# Autodesk Inventor assembly: motor_assembly
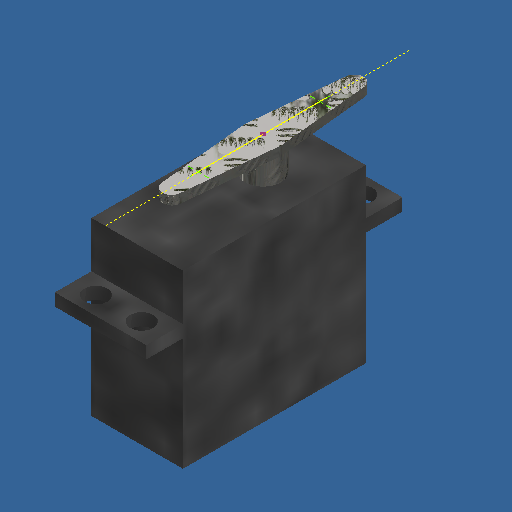
[picture p0: Inventor's stored thumbnail of the model, 512x512]
Saved by Autodesk Inventor 2025 (Build 290162000, 162)
## iProperties
Created: 2024-11-29
Part Number: motor_assembly
Document SubType Name: Assembly
Designer: Pauline Simonnet
Author: Pauline Simonnet
## Documents named in this file (3)
- C:\Users\Pauline Simonnet\Documents\ISAE SUPAERO\SupaeroMoon\MDRS\components\motor_assembly.iam
- C:\Users\Pauline Simonnet\Documents\ISAE SUPAERO\SupaeroMoon\MDRS\components\motor.ipt
- C:\Users\Pauline Simonnet\Documents\ISAE SUPAERO\SupaeroMoon\MDRS\components\motor_adaptator.ipt
## Components (2 placed, 2 different names)
1. motor:1 — Mate:1, Mate:2, Angle:1
2. motor_adaptator:1 — Mate:1, Mate:2, Angle:1
## Relationships (3: Mate 2, Angle 1)
- Mate:1: motor:1 ↔ motor_adaptator:1
- Mate:2: motor:1 ↔ motor_adaptator:1
- Angle:1 (0 deg): motor:1 ↔ motor_adaptator:1
